# Autodesk Inventor assembly: Assembly1
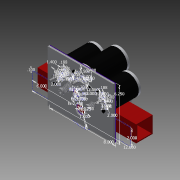
[picture p0: Inventor's stored thumbnail of the model, 180x180]
Saved by Autodesk Inventor 2013 (Build 170138000, 138)
## iProperties
Created: 2013-06-03
Part Number: Assembly1
Document SubType Name: Assembly
Designer: mvarma
Author: mvarma
## Documents named in this file (9)
- C:\Users\mvarma\Desktop\GRT 2013-2014 Gearbox\Mark 1\Assembly1.iam
- C:\Users\mvarma\Desktop\GRT 2013-2014 Gearbox\Mark 1\Frame Segment.ipt
- C:\Users\mvarma\Desktop\GRT 2013-2014 Gearbox\Mark 1\Cim Plate.ipt
- C:\Users\mvarma\Desktop\GRT 2013-2014 Gearbox\Mark 1\Motors\CIM Motor.ipt
- C:\Users\mvarma\Desktop\GRT 2013-2014 Gearbox\Mark 1\Motors\Mini CIM Motor.ipt
- C:\Users\mvarma\Desktop\GRT 2013-2014 Gearbox\Mark 1\Wheel Temp.ipt
- C:\Users\mvarma\Desktop\GRT 2013-2014 Gearbox\Mark 1\Bolts\Socket Head Cap Screw 10-32 Thread .500 Length.ipt
- C:\Users\mvarma\Desktop\GRT 2013-2014 Gearbox\Mark 1\Pulleys\16T 3mm GT2 - 8mm Key Broach.ipt
- C:\Users\mvarma\Desktop\GRT 2013-2014 Gearbox\Mark 1\Pulleys\19T 3mm GT2 - 8mm Key Broach.ipt
## Components (16 placed, 8 different names)
1. Frame Segment:1 — Mate:1, Angle:1, Mate:11
2. Cim Plate:1 — Mate:1, Angle:1, Mate:2, Mate:3, Mate:4, Mate:5, Mate:6, Mate:7, Mate:8, Mate:9, Mate:10, Mate:12, Mate:13, Mate:14, Mate:15, Mate:16, Mate:17, Mate:18, Mate:19, Mate:20, Mate:21, Mate:22, Mate:23
3. Wheel Temp:1 — Mate:11
4. 16T 3mm GT2 - 8mm Key Broach:1 — Mate:25, Flush:5, Mate:30
5. 16T 3mm GT2 - 8mm Key Broach:2 — Mate:24, Flush:1, Mate:28
6. 16T 3mm GT2 - 8mm Key Broach:3 — Mate:26, Flush:3
7. 19T 3mm GT2 - 8mm Key Broach:1 — Mate:29, Flush:4, Mate:30
8. CIM Motor:1 — Mate:3, Mate:4, Mate:5, Mate:25, Mate:29, Flush:4, Flush:5
9. CIM Motor:2 — Mate:2, Mate:6, Mate:7, Mate:24, Flush:1, Mate:28
10. Mini CIM Motor:1 — Mate:8, Mate:9, Mate:10, Mate:26, Flush:3
11. Socket Head Cap Screw 10-32 Thread .500 Length:1 — Mate:13, Mate:20
12. Socket Head Cap Screw 10-32 Thread .500 Length:2 — Mate:12, Mate:19
13. Socket Head Cap Screw 10-32 Thread .500 Length:3 — Mate:14, Mate:21
14. Socket Head Cap Screw 10-32 Thread .500 Length:4 — Mate:15, Mate:18
15. Socket Head Cap Screw 10-32 Thread .500 Length:5 — Mate:16, Mate:22
16. Socket Head Cap Screw 10-32 Thread .500 Length:6 — Mate:17, Mate:23
## Relationships (34: Mate 29, Flush 4, Angle 1)
- Mate:1: Frame Segment:1 ↔ Cim Plate:1
- Angle:1 (0 deg): Frame Segment:1 ↔ Cim Plate:1
- Mate:2: Cim Plate:1 ↔ CIM Motor:2
- Mate:3: Cim Plate:1 ↔ CIM Motor:1
- Mate:4: Cim Plate:1 ↔ CIM Motor:1
- Mate:5: Cim Plate:1 ↔ CIM Motor:1
- Mate:6: Cim Plate:1 ↔ CIM Motor:2
- Mate:7: Cim Plate:1 ↔ CIM Motor:2
- Mate:8: Cim Plate:1 ↔ Mini CIM Motor:1
- Mate:9: Cim Plate:1 ↔ Mini CIM Motor:1
- Mate:10: Cim Plate:1 ↔ Mini CIM Motor:1
- Mate:11: Frame Segment:1 ↔ Wheel Temp:1
- Mate:12: Cim Plate:1 ↔ Socket Head Cap Screw 10-32 Thread .500 Length:2
- Mate:13: Cim Plate:1 ↔ Socket Head Cap Screw 10-32 Thread .500 Length:1
- Mate:14: Cim Plate:1 ↔ Socket Head Cap Screw 10-32 Thread .500 Length:3
- Mate:15: Cim Plate:1 ↔ Socket Head Cap Screw 10-32 Thread .500 Length:4
- Mate:16: Cim Plate:1 ↔ Socket Head Cap Screw 10-32 Thread .500 Length:5
- Mate:17: Cim Plate:1 ↔ Socket Head Cap Screw 10-32 Thread .500 Length:6
- Mate:18: Cim Plate:1 ↔ Socket Head Cap Screw 10-32 Thread .500 Length:4
- Mate:19: Cim Plate:1 ↔ Socket Head Cap Screw 10-32 Thread .500 Length:2
- Mate:20: Cim Plate:1 ↔ Socket Head Cap Screw 10-32 Thread .500 Length:1
- Mate:21: Cim Plate:1 ↔ Socket Head Cap Screw 10-32 Thread .500 Length:3
- Mate:22: Cim Plate:1 ↔ Socket Head Cap Screw 10-32 Thread .500 Length:5
- Mate:23: Cim Plate:1 ↔ Socket Head Cap Screw 10-32 Thread .500 Length:6
- Mate:24: 16T 3mm GT2 - 8mm Key Broach:2 ↔ CIM Motor:2
- Flush:1: 16T 3mm GT2 - 8mm Key Broach:2 ↔ CIM Motor:2
- Mate:25: 16T 3mm GT2 - 8mm Key Broach:1 ↔ CIM Motor:1
- Mate:26: 16T 3mm GT2 - 8mm Key Broach:3 ↔ Mini CIM Motor:1
- Flush:3: 16T 3mm GT2 - 8mm Key Broach:3 ↔ Mini CIM Motor:1
- Mate:28: 16T 3mm GT2 - 8mm Key Broach:2 ↔ CIM Motor:2
- Mate:29: 19T 3mm GT2 - 8mm Key Broach:1 ↔ CIM Motor:1
- Flush:4: 19T 3mm GT2 - 8mm Key Broach:1 ↔ CIM Motor:1
- Flush:5: 16T 3mm GT2 - 8mm Key Broach:1 ↔ CIM Motor:1
- Mate:30: 16T 3mm GT2 - 8mm Key Broach:1 ↔ 19T 3mm GT2 - 8mm Key Broach:1
